# Autodesk Inventor assembly: universal_carriage_assembly
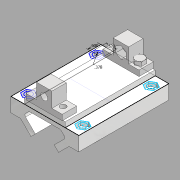
[picture p0: Inventor's stored thumbnail of the model, 180x180]
Saved by Autodesk Inventor 2020 (Build 240168000, 168)
## iProperties
Created: 2021-04-20
Part Number: universal_carriage_assembly
Document SubType Name: Assembly
Designer: griss
Author: griss
## Documents named in this file (6)
- C:\Users\griss\Documents\Inventor\CNC\y_axis_carriage\universal_carriage_assembly.iam
- C:\Users\griss\Documents\Inventor\CNC\y_axis_carriage\universal_carriage.ipt
- C:\Users\griss\Documents\Inventor\CNC\connections\608-2RS_BALL BEARING.ipt
- C:\Users\griss\Documents\Inventor\CNC\connections\91309A583_LOW-STRENGTH ZINC-PLATED STEEL CAP SCREW.ipt
- C:\Users\griss\Documents\Inventor\CNC\y_axis_lead_screw_insert.ipt
- C:\Users\griss\Documents\Inventor\CNC\connections\90473A030_LOW-STRENGTH STEEL HEX NUT.ipt
## Components (15 placed, 5 different names)
1. universal_carriage:1 — Mate:1, Mate:2, Mate:3, Mate:4, Mate:5, Mate:6, Mate:7, Mate:8, Mate:11, Mate:17, Mate:18, Mate:19, Mate:20, Mate:21, Mate:22, Mate:24, Mate:28, Mate:30
2. 608-2RS_BALL BEARING:1 — Mate:7, Mate:8, Mate:15, Mate:16
3. 608-2RS_BALL BEARING:2 — Mate:3, Mate:4, Mate:12
4. 608-2RS_BALL BEARING:3 — Mate:1, Mate:2, Mate:9, Mate:10
5. 608-2RS_BALL BEARING:4 — Mate:5, Mate:6, Mate:13, Mate:14
6. 91309A583_LOW-STRENGTH ZINC-PLATED STEEL CAP SCREW:1 — Mate:9, Mate:10
7. 91309A583_LOW-STRENGTH ZINC-PLATED STEEL CAP SCREW:2 — Mate:13, Mate:14, Mate:29
8. 91309A583_LOW-STRENGTH ZINC-PLATED STEEL CAP SCREW:3 — Mate:11, Mate:12
9. 91309A583_LOW-STRENGTH ZINC-PLATED STEEL CAP SCREW:4 — Mate:15, Mate:16, Mate:27
10. y_axis_lead_screw_insert:1 — Mate:17, Mate:18, Mate:19, Mate:23, Mate:26
11. y_axis_lead_screw_insert:2 — Mate:20, Mate:21, Mate:22
12. 91309A583_LOW-STRENGTH ZINC-PLATED STEEL CAP SCREW:5 — Mate:23, Mate:25, Mate:26
13. 90473A030_LOW-STRENGTH STEEL HEX NUT:1 — Mate:27, Mate:28
14. 90473A030_LOW-STRENGTH STEEL HEX NUT:2 — Mate:24, Mate:25
15. 90473A030_LOW-STRENGTH STEEL HEX NUT:3 — Mate:29, Mate:30
## Relationships (30: Mate 30)
- Mate:1: universal_carriage:1 ↔ 608-2RS_BALL BEARING:3
- Mate:2: universal_carriage:1 ↔ 608-2RS_BALL BEARING:3
- Mate:3: universal_carriage:1 ↔ 608-2RS_BALL BEARING:2
- Mate:4: universal_carriage:1 ↔ 608-2RS_BALL BEARING:2
- Mate:5: universal_carriage:1 ↔ 608-2RS_BALL BEARING:4
- Mate:6: universal_carriage:1 ↔ 608-2RS_BALL BEARING:4
- Mate:7: universal_carriage:1 ↔ 608-2RS_BALL BEARING:1
- Mate:8: universal_carriage:1 ↔ 608-2RS_BALL BEARING:1
- Mate:9: 608-2RS_BALL BEARING:3 ↔ 91309A583_LOW-STRENGTH ZINC-PLATED STEEL CAP SCREW:1
- Mate:10: 608-2RS_BALL BEARING:3 ↔ 91309A583_LOW-STRENGTH ZINC-PLATED STEEL CAP SCREW:1
- Mate:11: universal_carriage:1 ↔ 91309A583_LOW-STRENGTH ZINC-PLATED STEEL CAP SCREW:3
- Mate:12: 608-2RS_BALL BEARING:2 ↔ 91309A583_LOW-STRENGTH ZINC-PLATED STEEL CAP SCREW:3
- Mate:13: 608-2RS_BALL BEARING:4 ↔ 91309A583_LOW-STRENGTH ZINC-PLATED STEEL CAP SCREW:2
- Mate:14: 608-2RS_BALL BEARING:4 ↔ 91309A583_LOW-STRENGTH ZINC-PLATED STEEL CAP SCREW:2
- Mate:15: 608-2RS_BALL BEARING:1 ↔ 91309A583_LOW-STRENGTH ZINC-PLATED STEEL CAP SCREW:4
- Mate:16: 608-2RS_BALL BEARING:1 ↔ 91309A583_LOW-STRENGTH ZINC-PLATED STEEL CAP SCREW:4
- Mate:17: universal_carriage:1 ↔ y_axis_lead_screw_insert:1
- Mate:18: universal_carriage:1 ↔ y_axis_lead_screw_insert:1
- Mate:19: universal_carriage:1 ↔ y_axis_lead_screw_insert:1
- Mate:20: universal_carriage:1 ↔ y_axis_lead_screw_insert:2
- Mate:21: universal_carriage:1 ↔ y_axis_lead_screw_insert:2
- Mate:22: universal_carriage:1 ↔ y_axis_lead_screw_insert:2
- Mate:23: y_axis_lead_screw_insert:1 ↔ 91309A583_LOW-STRENGTH ZINC-PLATED STEEL CAP SCREW:5
- Mate:24: universal_carriage:1 ↔ 90473A030_LOW-STRENGTH STEEL HEX NUT:2
- Mate:25: 91309A583_LOW-STRENGTH ZINC-PLATED STEEL CAP SCREW:5 ↔ 90473A030_LOW-STRENGTH STEEL HEX NUT:2
- Mate:26: y_axis_lead_screw_insert:1 ↔ 91309A583_LOW-STRENGTH ZINC-PLATED STEEL CAP SCREW:5
- Mate:27: 91309A583_LOW-STRENGTH ZINC-PLATED STEEL CAP SCREW:4 ↔ 90473A030_LOW-STRENGTH STEEL HEX NUT:1
- Mate:28: universal_carriage:1 ↔ 90473A030_LOW-STRENGTH STEEL HEX NUT:1
- Mate:29: 91309A583_LOW-STRENGTH ZINC-PLATED STEEL CAP SCREW:2 ↔ 90473A030_LOW-STRENGTH STEEL HEX NUT:3
- Mate:30: universal_carriage:1 ↔ 90473A030_LOW-STRENGTH STEEL HEX NUT:3
